# Autodesk Inventor assembly: GreyT Claw 2 Wheel Configurations
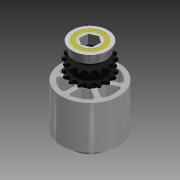
[picture p0: Inventor's stored thumbnail of the model, 180x180]
Saved by Autodesk Inventor 2022 (Build 260153000, 153)
## iProperties
Created: 2022-01-08
Part Number: GreyT Claw 2 Wheel Configurations
Document SubType Name: Assembly
## iProperties of the stored document MemberDocs/x2srp4ngiLs1iruelMuc3cy3v1a
Created: 2022-01-08
Part Number: GreyT Claw 2 Wheel Configurations
Document SubType Name: Assembly
Mass: 230.119 g
Surface Area: 693.144 cm^2
Volume: 122.266 cm^3
Density: 1.88213 g/cm^3
## iProperties of the stored document MemberDocs/x2n4c4ajrDs32nofjKwl10j514h
Created: 2022-01-08
Part Number: GreyT Claw 2 Wheel Configurations
Document SubType Name: Assembly
Mass: 158.965 g
Surface Area: 390.851 cm^2
Volume: 68.8837 cm^3
Density: 2.30773 g/cm^3
## iProperties of the stored document MemberDocs/xL1ddyaiwHcvpx5fjBcot5ityDb
Created: 2022-01-08
Part Number: GreyT Claw 2 Wheel Configurations
Document SubType Name: Assembly
Mass: 250.311 g
Surface Area: 625.895 cm^2
Volume: 121.028 cm^3
Density: 2.0682 g/cm^3
## iProperties of the stored document MemberDocs/xDs45beceD0mblsaiTrand0jePd
Created: 2022-01-08
Part Number: GreyT Claw 2 Wheel Configurations
Document SubType Name: Assembly
Mass: 288.634 g
Surface Area: 752.073 cm^2
Volume: 159.351 cm^3
Density: 1.81131 g/cm^3
## iProperties of the stored document MemberDocs/xS142r35mFk55cswpX2krkrcw0c
Created: 2022-01-08
Part Number: GreyT Claw 2 Wheel Configurations
Document SubType Name: Assembly
Mass: 489.208 g
Surface Area: 1412.13 cm^2
Volume: 303.111 cm^3
Density: 1.61396 g/cm^3
## Documents named in this file (35)
- C:\Users\Cal\Desktop\Robotics\Design\Collaborative\Collaborative Parts Library\Standard Custom Parts\Plates\GreyT Claw 2 Configurations\GreyT Claw 2 Wheel Configurations.iam
- C:\Users\Cal\Desktop\Robotics\Design\Collaborative\Collaborative Parts Library\Power Transfer\Bearings and Bushings\Bearings\FR8 Hex.ipt
- C:\Users\Cal\Desktop\Robotics\Design\Collaborative\Collaborative Parts Library\Power Transfer\Bearings and Bushings\Bearings.ipt
- C:\Users\Cal\Desktop\Robotics\Design\Collaborative\Collaborative Parts Library\Power Transfer\Sprockets\Sprockets\VexPro 16T 25 Chain 500 Hex Bore Double Sprocket.ipt
- C:\Users\Cal\Desktop\Robotics\Design\Collaborative\Collaborative Parts Library\Power Transfer\Sprockets\VexPro Sprockets.ipt
- C:\Users\Cal\Desktop\Robotics\Design\Collaborative\Collaborative Parts Library\Hardware\Spacers\Spacers & Standoffs\VexPro 500 Hex Spacer 0.125in.ipt
- C:\Users\Cal\Desktop\Robotics\Design\Collaborative\Collaborative Parts Library\Hardware\Spacers\Spacers & Standoffs.ipt
- C:\Users\Cal\Desktop\Robotics\Design\Collaborative\Collaborative Parts Library\Wheels\Compliant Wheel Generator\2 in 30A .5 in Hex Compliant Wheel VEX.ipt
- C:\Users\Cal\Desktop\Robotics\Design\Collaborative\Collaborative Parts Library\Wheels\Compliant Wheel Generator.ipt
- C:\Users\Cal\Desktop\Robotics\Design\Collaborative\Collaborative Parts Library\Power Transfer\Hubs (Hex and Key)\VersaHub .500 Hex (Plastic).ipt
- C:\Users\Cal\Desktop\Robotics\Design\Collaborative\Collaborative Parts Library\Hardware\Fasteners\Machine Screws\10-32 UNFx1.25 Button Head Cap Screw.ipt
- C:\Users\Cal\Desktop\Robotics\Design\Collaborative\Collaborative Parts Library\Hardware\Fasteners\Machine Screws.ipt
- C:\Users\Cal\Desktop\Robotics\Design\Collaborative\Collaborative Parts Library\Wheels\Compliant Wheel Generator\3 in 30A 1.125 in Hex Compliant Wheel VEX.ipt
- C:\Users\Cal\Desktop\Robotics\Design\Collaborative\Collaborative Parts Library\Wheels\Compliant Wheels\Compliant Wheel Generator.ipt
- C:\Users\Cal\Desktop\Robotics\Design\Collaborative\Collaborative Parts Library\Hardware\Spacers\Spacers & Standoffs\VexPro 500 Hex Spacer 0.5in.ipt
- C:\Users\Cal\Desktop\Robotics\Design\Collaborative\Collaborative Parts Library\Hardware\Spacers\Spacers & Standoffs\VexPro 500 Hex Spacer 1in.ipt
- C:\Users\Cal\Desktop\Robotics\Design\Collaborative\Collaborative Parts Library\Wheels\Compliant Wheels\Compliant Wheel Generator\2 in od .5 in Hex VEX 30A.ipt
- C:\Users\Cal\Desktop\Robotics\Design\Collaborative\Collaborative Parts Library\Standard Custom Parts\Plates\GreyT Claw 2 Configurations\GreyT Claw 2 Wheel Shaft.ipt
- C:\Users\Cal\Desktop\Robotics\Design\Collaborative\Collaborative Parts Library\Wheels\Compliant Wheels\Compliant Wheel Generator\3 in od 1.125 in Round Bore VEX 30A.ipt
- E:\Collaborative Robots\Collaborative Part Library\Power Transfer\Bearings and Bushings\Bearings\FR8 Hex.ipt
- E:\Collaborative Robots\Collaborative Part Library\Power Transfer\Sprockets\Sprockets\VexPro 16T 25 Chain 500 Hex Bore Double Sprocket.ipt
- E:\Collaborative Robots\Collaborative Part Library\Hardware\Spacers\Spacers & Standoffs\VexPro 500 Hex Spacer 0.125in.ipt
- E:\Collaborative Robots\Collaborative Part Library\Hardware\Spacers\Spacers & Standoffs.ipt
- E:\Collaborative Robots\Collaborative Part Library\Wheels\Compliant Wheels\Compliant Wheel Generator.ipt
- E:\Collaborative Robots\Collaborative Part Library\Power Transfer\Hubs (Hex and Key)\VersaHub .500 Hex (Plastic).ipt
- E:\Collaborative Robots\Collaborative Part Library\Hardware\Fasteners\Machine Screws\10-32 UNFx1.25 Button Head Cap Screw.ipt
- E:\Collaborative Robots\Collaborative Part Library\Hardware\Spacers\Spacers & Standoffs\VexPro 500 Hex Spacer 0.5in.ipt
- E:\Collaborative Robots\Collaborative Part Library\Hardware\Spacers\Spacers & Standoffs\VexPro 500 Hex Spacer 1in.ipt
- E:\Collaborative Robots\Collaborative Part Library\Wheels\Compliant Wheels\Compliant Wheel Generator\2 in od .5 in Hex VEX 30A.ipt
- E:\Collaborative Robots\Collaborative Part Library\Standard Custom Parts\Plates\GreyT Claw 2 Configurations\GreyT Claw 2 Wheel Shaft.ipt
- E:\Collaborative Robots\Collaborative Part Library\Wheels\Compliant Wheels\Compliant Wheel Generator\3 in od 1.125 in Round Bore VEX 30A.ipt
- C:\Users\Cal\Desktop\Robotics\Design\Collaborative\Collaborative Parts Library\Hardware\Spacers\Spacers & Standoffs\VexPro 500 Hex Spacer 0.25in.ipt
- C:\Users\Cal\Desktop\Robotics\Design\Collaborative\Collaborative Parts Library\Wheels\Compliant Wheels\Compliant Wheel Generator\4 in od 1.125 in Round Bore VEX 30A.ipt
- E:\Collaborative Robots\Collaborative Part Library\Hardware\Spacers\Spacers & Standoffs\VexPro 500 Hex Spacer 0.25in.ipt
- E:\Collaborative Robots\Collaborative Part Library\Wheels\Compliant Wheels\Compliant Wheel Generator\4 in od 1.125 in Round Bore VEX 30A.ipt
## Components (18 placed, 7 different names)
1. FR8 Hex:1 — Mate:1, Symmetry:1, Mate:2, Mate:3, Flush:1, Flush:2, Insert:1
2. FR8 Hex:2 — Mate:1, Symmetry:1, Mate:3, Flush:1, Insert:4, Insert:9, Mate:7, Mate:9
3. VexPro 16T 25 Chain 500 Hex Bore Double Sprocket:1 — Flush:2, Insert:2, Insert:3
4. VexPro 500 Hex Spacer 0.125in:1 — Insert:1, Insert:2
5. VexPro 500 Hex Spacer 0.125in:2 — Insert:3, Mate:6
6. 2 in 30A .5 in Hex Compliant Wheel VEX:1 — Insert:6
7. 2 in 30A .5 in Hex Compliant Wheel VEX:2 — Insert:5, Insert:6
8. 2 in 30A .5 in Hex Compliant Wheel VEX:3 — Insert:4, Insert:5
9. 3 in 30A 1.125 in Hex Compliant Wheel VEX:4 — Insert:7, Insert:8, Mate:5, Mate:7, Mate:8, Mate:9
10. VersaHub .500 Hex (Plastic):1 — Insert:7, Mate:4, Mate:6
11. VersaHub .500 Hex (Plastic):2 — Insert:8, Mate:5, Insert:10, Insert:11, Insert:12, Insert:13, Insert:14, Insert:15
12. VexPro 500 Hex Spacer 0.125in:4 — Insert:9
13. 10-32 UNFx1.25 Button Head Cap Screw:1 — Insert:10, Mate:4, Mate:8
14. 10-32 UNFx1.25 Button Head Cap Screw:2 — Insert:11
15. 10-32 UNFx1.25 Button Head Cap Screw:3 — Insert:12
16. 10-32 UNFx1.25 Button Head Cap Screw:4 — Insert:13
17. 10-32 UNFx1.25 Button Head Cap Screw:5 — Insert:14
18. 10-32 UNFx1.25 Button Head Cap Screw:6 — Insert:15
## Relationships (27: Insert 15, Mate 9, Flush 2, Symmetry 1)
- Mate:1: FR8 Hex:1 ↔ FR8 Hex:2
- Symmetry:1: FR8 Hex:1 ↔ FR8 Hex:2
- Mate:2: FR8 Hex:1
- Mate:3 (73.025 mm): FR8 Hex:1 ↔ FR8 Hex:2
- Flush:1: FR8 Hex:1 ↔ FR8 Hex:2
- Flush:2: FR8 Hex:1 ↔ VexPro 16T 25 Chain 500 Hex Bore Double Sprocket:1
- Insert:1: FR8 Hex:1 ↔ VexPro 500 Hex Spacer 0.125in:1
- Insert:2: VexPro 16T 25 Chain 500 Hex Bore Double Sprocket:1 ↔ VexPro 500 Hex Spacer 0.125in:1
- Insert:3: VexPro 16T 25 Chain 500 Hex Bore Double Sprocket:1 ↔ VexPro 500 Hex Spacer 0.125in:2
- Insert:4: FR8 Hex:2 ↔ 2 in 30A .5 in Hex Compliant Wheel VEX:3
- Insert:5: 2 in 30A .5 in Hex Compliant Wheel VEX:2 ↔ 2 in 30A .5 in Hex Compliant Wheel VEX:3
- Insert:6: 2 in 30A .5 in Hex Compliant Wheel VEX:1 ↔ 2 in 30A .5 in Hex Compliant Wheel VEX:2
- Insert:7: 3 in 30A 1.125 in Hex Compliant Wheel VEX:4 ↔ VersaHub .500 Hex (Plastic):1
- Mate:4: VersaHub .500 Hex (Plastic):1 ↔ 10-32 UNFx1.25 Button Head Cap Screw:1
- Insert:8: 3 in 30A 1.125 in Hex Compliant Wheel VEX:4 ↔ VersaHub .500 Hex (Plastic):2
- Mate:5: 3 in 30A 1.125 in Hex Compliant Wheel VEX:4 ↔ VersaHub .500 Hex (Plastic):2
- Mate:6: VexPro 500 Hex Spacer 0.125in:2 ↔ VersaHub .500 Hex (Plastic):1
- Insert:9: FR8 Hex:2 ↔ VexPro 500 Hex Spacer 0.125in:4
- Insert:10: VersaHub .500 Hex (Plastic):2 ↔ 10-32 UNFx1.25 Button Head Cap Screw:1
- Insert:11: VersaHub .500 Hex (Plastic):2 ↔ 10-32 UNFx1.25 Button Head Cap Screw:2
- Insert:12: VersaHub .500 Hex (Plastic):2 ↔ 10-32 UNFx1.25 Button Head Cap Screw:3
- Insert:13: VersaHub .500 Hex (Plastic):2 ↔ 10-32 UNFx1.25 Button Head Cap Screw:4
- Insert:14: VersaHub .500 Hex (Plastic):2 ↔ 10-32 UNFx1.25 Button Head Cap Screw:5
- Insert:15: VersaHub .500 Hex (Plastic):2 ↔ 10-32 UNFx1.25 Button Head Cap Screw:6
- Mate:7: FR8 Hex:2 ↔ 3 in 30A 1.125 in Hex Compliant Wheel VEX:4
- Mate:8: 3 in 30A 1.125 in Hex Compliant Wheel VEX:4 ↔ 10-32 UNFx1.25 Button Head Cap Screw:1
- Mate:9: FR8 Hex:2 ↔ 3 in 30A 1.125 in Hex Compliant Wheel VEX:4
